# Autodesk Inventor assembly: Housing
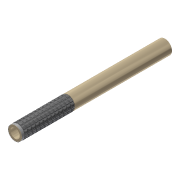
[picture p0: Inventor's stored thumbnail of the model, 180x180]
Saved by Autodesk Inventor 2022 (Build 260148000, 148)
## iProperties
Created: 2009-06-23
Part Number: Housing
Document SubType Name: Assembly
Designer: jmacmillan
Author: jmacmillan
## Documents named in this file (4)
- C:\Autodesk Inventor 2022 Advanced Assembly Modeling Practice Files\Mechanical_Pencil_Shrinkwrap\Housing.iam
- C:\Autodesk Inventor 2022 Advanced Assembly Modeling Practice Files\Mechanical_Pencil_Shrinkwrap\Sleeve.ipt
- C:\Autodesk Inventor 2022 Advanced Assembly Modeling Practice Files\Mechanical_Pencil_Shrinkwrap\Grip.ipt
- C:\Autodesk Inventor 2022 Advanced Assembly Modeling Practice Files\Mechanical_Pencil_Shrinkwrap\Ring.ipt
## Components (3 placed, 3 different names)
1. Sleeve:1
2. Ring:1
3. Grip:1
## Relationships (2: Insert 2)
- [Insert]: Sleeve:1 ↔ Grip:1
- [Insert]: Ring:1 ↔ Grip:1
